# Autodesk Inventor assembly: ALU
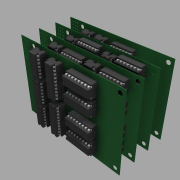
[picture p0: Inventor's stored thumbnail of the model, 180x180]
Saved by Autodesk Inventor 2019.4 (Build 234330000, 330)
## iProperties
Created: 2021-09-13
Part Number: ALU
Document SubType Name: Assembly
Designer: erics
Mass: 50.5563 g
Surface Area: 1575.73 cm^2
Volume: 50.5563 cm^3
Density: 1 g/cm^3
Author: erics
## Documents named in this file (5)
- D:\Users\erics\Documents\16B\Mechanical\ALU.iam
- D:\Users\erics\Documents\16B\ALU_Adder_ZF\ALU_Adder_ZF.iam
- D:\Users\erics\Documents\16B\ALU_AND_OR\ALU_AND_OR.iam
- D:\Users\erics\Documents\16B\ALU_Shifter\ALU_Shifter.iam
- D:\Users\erics\Documents\16B\ALU_XOR_ONES\ALU_XOR_ONES.iam
## Components (4 placed, 4 different names)
1. ALU_Adder_ZF:1 [sub-assembly] — Mate:1, Mate:2, Mate:5, Mate:6
2. ALU_AND_OR:1 [sub-assembly] — Mate:1, Mate:2, Mate:3, Mate:5, Mate:6, Mate:7, Mate:8
3. ALU_Shifter:1 [sub-assembly] — Mate:3, Mate:4, Mate:7, Mate:8, Mate:9, Mate:10
4. ALU_XOR_ONES:1 [sub-assembly] — Mate:4, Mate:9, Mate:10
## Relationships (10: Mate 10)
- Mate:1: ALU_Adder_ZF:1 ↔ ALU_AND_OR:1
- Mate:2 (14 mm): ALU_Adder_ZF:1 ↔ ALU_AND_OR:1
- Mate:3 (14 mm): ALU_AND_OR:1 ↔ ALU_Shifter:1
- Mate:4 (14 mm): ALU_Shifter:1 ↔ ALU_XOR_ONES:1
- Mate:5: ALU_Adder_ZF:1 ↔ ALU_AND_OR:1
- Mate:6: ALU_Adder_ZF:1 ↔ ALU_AND_OR:1
- Mate:7: ALU_AND_OR:1 ↔ ALU_Shifter:1
- Mate:8: ALU_AND_OR:1 ↔ ALU_Shifter:1
- Mate:9: ALU_Shifter:1 ↔ ALU_XOR_ONES:1
- Mate:10: ALU_Shifter:1 ↔ ALU_XOR_ONES:1
## Named parameters: Spacing = 14 mm
